# Autodesk Inventor assembly: Piston Feed Platform assy
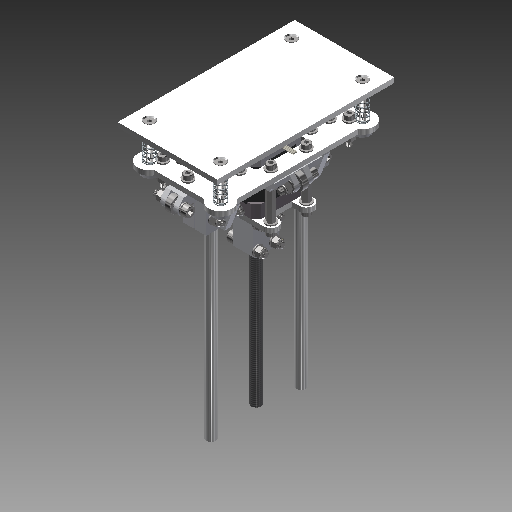
[picture p0: Inventor's stored thumbnail of the model, 512x512]
Saved by Autodesk Inventor 2018 (Build 220112000, 112)
## iProperties
Created: 2017-09-29
Part Number: Piston Feed Platform assy
Document SubType Name: Assembly
Designer: Gabriel Smolnycki
Author: Gabriel Smolnycki
## Documents named in this file (15)
- E:\planb\mechanics\Subassemblies\Piston Feed Platform assy.iam
- E:\planb\mechanics\Piston\Piston Feed Frame.ipt
- E:\planb\mechanics\Subassemblies\Piston Guide assy.iam
- E:\planb\mechanics\Hardware\M4x20 SS SHCS.ipt
- E:\planb\mechanics\Hardware\M4 SS Washer.ipt
- E:\planb\mechanics\Hardware\M4 SS Locknut.ipt
- E:\planb\mechanics\Subassemblies\Piston Wall Guide Wide assy.iam
- E:\planb\mechanics\Subassemblies\Piston Wall Guide Small assy.iam
- E:\planb\mechanics\Piston\Piston Nut Trap.ipt
- E:\planb\mechanics\Piston\Piston Feed Surface.ipt
- E:\planb\mechanics\Hardware\0.375x1.000 Steel Spring (9657K306).ipt
- E:\planb\mechanics\Hardware\M4x40 SS FHSS.ipt
- E:\planb\mechanics\Subassemblies\Piston Motor Holder assy.iam
- E:\planb\mechanics\Hardware\M4x25 SS Standoff FF (94868A045).ipt
- E:\planb\mechanics\Hardware\M4x12 SS SHCS.ipt
## Components (109 placed, 14 different names)
1. Piston Feed Frame:1 — Insert:1, Insert:2, Insert:3, Insert:4, Insert:5, Insert:6, Insert:7, Insert:8, Insert:9, Insert:10, Insert:11, Insert:12, Insert:37, Insert:38, Insert:39, Insert:40, Flush:1, Mate:1, Tangent:1, Mate:4, Flush:2, Tangent:2, Insert:53, Mate:7, Insert:54, Mate:8, Insert:56, Insert:60, Insert:63, Insert:64, Insert:65, Insert:78, Insert:79, Insert:80, Insert:81, Insert:82, Insert:83, Insert:84, Insert:85, Insert:86, Mate:29, Insert:87, Insert:88
2. Piston Guide assy:1 [sub-assembly] — Insert:3, Insert:4, Insert:15, Insert:16, Insert:19, Insert:20
3. Piston Guide assy:2 [sub-assembly] — Insert:1, Insert:2, Insert:13, Insert:14, Insert:17, Insert:18
4. M4x20 SS SHCS:1 — Insert:36
5. M4x20 SS SHCS:2 — Insert:35
6. M4x20 SS SHCS:3 — Insert:32
7. M4x20 SS SHCS:4 — Insert:31
8. M4x20 SS SHCS:5 — Insert:34
9. M4x20 SS SHCS:6 — Insert:33
10. M4x20 SS SHCS:7 — Insert:30
11. M4x20 SS SHCS:8 — Insert:29
12. M4 SS Washer:1 — Insert:18, Insert:24
13. M4 SS Washer:2 — Insert:15, Insert:26
14. M4 SS Washer:3 — Insert:9, Insert:33
15. M4 SS Washer:4 — Insert:7, Insert:35
16. M4 SS Washer:5 — Insert:8, Insert:36
17. M4 SS Washer:6 — Insert:11, Insert:31
18. M4 SS Washer:7 — Insert:16, Insert:25
19. M4 SS Washer:8 — Insert:19, Insert:28
20. M4 SS Washer:9 — Insert:20, Insert:27
21. M4 SS Washer:10 — Insert:17, Insert:22
22. M4 SS Washer:11 — Insert:12, Insert:32
23. M4 SS Washer:12 — Insert:6, Insert:30
24. M4 SS Washer:13 — Insert:10, Insert:34
25. M4 SS Washer:14 — Insert:13, Insert:23
26. M4 SS Washer:15 — Insert:14, Insert:21
27. M4 SS Washer:16 — Insert:5, Insert:29
28. M4 SS Locknut:1 — Insert:21
29. M4 SS Locknut:2 — Insert:22
30. M4 SS Locknut:3 — Insert:24
31. M4 SS Locknut:4 — Insert:23
32. M4 SS Locknut:5 — Insert:28
33. M4 SS Locknut:6 — Insert:27
34. M4 SS Locknut:7 — Insert:26
35. M4 SS Locknut:8 — Insert:25
36. Piston Wall Guide Wide assy:1 [sub-assembly] — Mate:4, Flush:2, Tangent:2, Mate:5, Mate:6
37. Piston Wall Guide Wide assy:2 [sub-assembly] — Flush:1, Mate:1, Tangent:1, Mate:2, Mate:3
38. M4 SS Washer:17 — Mate:5, Insert:92
39. M4 SS Washer:18 — Mate:6, Insert:91
40. M4 SS Washer:19 — Insert:40
41. M4 SS Washer:20 — Insert:39
42. M4 SS Washer:21 — Mate:2, Insert:89
43. M4 SS Washer:22 — Mate:3, Insert:90
44. M4 SS Washer:23 — Insert:38
45. M4 SS Washer:24 — Insert:37
46. M4x20 SS SHCS:9
47. M4x20 SS SHCS:10
48. M4x20 SS SHCS:11
49. M4x20 SS SHCS:12
50. Piston Wall Guide Small assy:1 [sub-assembly] — Insert:54, Mate:8, Insert:55
51. Piston Wall Guide Small assy:2 [sub-assembly] — Insert:53, Mate:7, Insert:59
52. M4 SS Washer:25 — Insert:60, Insert:61
53. M4 SS Washer:26 — Insert:59, Insert:62
54. M4 SS Washer:27 — Insert:56, Insert:57
55. M4 SS Washer:28 — Insert:55, Insert:58
56. M4 SS Locknut:13 — Insert:62
57. M4 SS Locknut:14 — Insert:58
58. M4x20 SS SHCS:13 — Insert:57
59. M4x20 SS SHCS:14 — Insert:61
60. Piston Nut Trap:1 — Mate:9, Flush:3, Mate:10, Insert:63, Insert:66
61. M4 SS Locknut:15 — Insert:67
62. M4 SS Locknut:16 — Mate:9, Flush:3, Mate:10, Insert:64
63. M4 SS Washer:29 — Insert:66, Insert:67
64. M4 SS Washer:30 — Insert:65, Insert:68
65. M4x20 SS SHCS:15 — Insert:68
66. Piston Nut Trap:2 — Insert:80
67. M4 SS Locknut:17
68. M4 SS Locknut:18 — Insert:79
69. M4 SS Washer:31
70. M4 SS Washer:32 — Insert:78
71. M4x20 SS SHCS:16
72. Piston Nut Trap:3 — Insert:82
73. M4 SS Locknut:19
74. M4 SS Locknut:20 — Insert:83
75. M4 SS Washer:33
76. M4 SS Washer:34 — Insert:81
77. M4x20 SS SHCS:17
78. Piston Nut Trap:4 — Insert:85
79. M4 SS Locknut:21
80. M4 SS Locknut:22 — Insert:86
81. M4 SS Washer:35
82. M4 SS Washer:36 — Insert:84
83. M4x20 SS SHCS:18
84. Piston Feed Surface:1 — Mate:17, Mate:18, Mate:19, Mate:20, Mate:21, Mate:22, Mate:23, Mate:24
85. 0.375x1.000 Steel Spring (9657K306):1 — Mate:24, Mate:25
86. 0.375x1.000 Steel Spring (9657K306):2 — Mate:23, Mate:26, Mate:29
87. 0.375x1.000 Steel Spring (9657K306):3 — Mate:22, Mate:27
88. 0.375x1.000 Steel Spring (9657K306):4 — Mate:21, Mate:28
89. M4x40 SS FHSS:1 — Mate:20, Mate:25
90. M4x40 SS FHSS:2 — Mate:19, Mate:26, Insert:88
91. M4x40 SS FHSS:3 — Mate:18, Mate:27, Insert:87
92. M4x40 SS FHSS:4 — Mate:17, Mate:28
93. Piston Motor Holder assy:1 [sub-assembly] — Insert:93, Insert:94, Insert:95, Insert:96, Insert:97, Insert:98, Insert:99, Insert:100
94. M4x25 SS Standoff FF (94868A045):1 — Insert:89, Insert:105
95. M4x25 SS Standoff FF (94868A045):2 — Insert:90
96. M4x25 SS Standoff FF (94868A045):3 — Insert:91, Insert:106
97. M4x25 SS Standoff FF (94868A045):4 — Insert:92
98. M4 SS Washer:37 — Insert:99, Insert:106
99. M4 SS Washer:38 — Insert:97
100. M4 SS Washer:39 — Insert:95, Insert:102
101. M4 SS Washer:40 — Insert:93, Insert:104
102. M4 SS Washer:41 — Insert:100, Insert:105
103. M4 SS Washer:42 — Insert:98
104. M4 SS Washer:43 — Insert:96, Insert:101
105. M4 SS Washer:44 — Insert:94, Insert:103
106. M4x12 SS SHCS:1 — Insert:104
107. M4x12 SS SHCS:2 — Insert:103
108. M4x12 SS SHCS:3 — Insert:102
109. M4x12 SS SHCS:4 — Insert:101
## Relationships (139: Insert 102, Mate 29, Flush 6, Tangent 2)
- Insert:1: Piston Feed Frame:1 ↔ Piston Guide assy:2
- Insert:2: Piston Feed Frame:1 ↔ Piston Guide assy:2
- Insert:3: Piston Feed Frame:1 ↔ Piston Guide assy:1
- Insert:4: Piston Feed Frame:1 ↔ Piston Guide assy:1
- Insert:5: Piston Feed Frame:1 ↔ M4 SS Washer:16
- Insert:6: Piston Feed Frame:1 ↔ M4 SS Washer:12
- Insert:7: Piston Feed Frame:1 ↔ M4 SS Washer:4
- Insert:8: Piston Feed Frame:1 ↔ M4 SS Washer:5
- Insert:9: Piston Feed Frame:1 ↔ M4 SS Washer:3
- Insert:10: Piston Feed Frame:1 ↔ M4 SS Washer:13
- Insert:11: Piston Feed Frame:1 ↔ M4 SS Washer:6
- Insert:12: Piston Feed Frame:1 ↔ M4 SS Washer:11
- Insert:13: Piston Guide assy:2 ↔ M4 SS Washer:14
- Insert:14: Piston Guide assy:2 ↔ M4 SS Washer:15
- Insert:15: Piston Guide assy:1 ↔ M4 SS Washer:2
- Insert:16: Piston Guide assy:1 ↔ M4 SS Washer:7
- Insert:17: Piston Guide assy:2 ↔ M4 SS Washer:10
- Insert:18: Piston Guide assy:2 ↔ M4 SS Washer:1
- Insert:19: Piston Guide assy:1 ↔ M4 SS Washer:8
- Insert:20: Piston Guide assy:1 ↔ M4 SS Washer:9
- Insert:21: M4 SS Washer:15 ↔ M4 SS Locknut:1
- Insert:22: M4 SS Washer:10 ↔ M4 SS Locknut:2
- Insert:23: M4 SS Washer:14 ↔ M4 SS Locknut:4
- Insert:24: M4 SS Washer:1 ↔ M4 SS Locknut:3
- Insert:25: M4 SS Washer:7 ↔ M4 SS Locknut:8
- Insert:26: M4 SS Washer:2 ↔ M4 SS Locknut:7
- Insert:27: M4 SS Washer:9 ↔ M4 SS Locknut:6
- Insert:28: M4 SS Washer:8 ↔ M4 SS Locknut:5
- Insert:29: M4x20 SS SHCS:8 ↔ M4 SS Washer:16
- Insert:30: M4x20 SS SHCS:7 ↔ M4 SS Washer:12
- Insert:31: M4x20 SS SHCS:4 ↔ M4 SS Washer:6
- Insert:32: M4x20 SS SHCS:3 ↔ M4 SS Washer:11
- Insert:33: M4x20 SS SHCS:6 ↔ M4 SS Washer:3
- Insert:34: M4x20 SS SHCS:5 ↔ M4 SS Washer:13
- Insert:35: M4x20 SS SHCS:2 ↔ M4 SS Washer:4
- Insert:36: M4x20 SS SHCS:1 ↔ M4 SS Washer:5
- Insert:37: Piston Feed Frame:1 ↔ M4 SS Washer:24
- Insert:38: Piston Feed Frame:1 ↔ M4 SS Washer:23
- Insert:39: Piston Feed Frame:1 ↔ M4 SS Washer:20
- Insert:40: Piston Feed Frame:1 ↔ M4 SS Washer:19
- Flush:1 (0.825 mm): Piston Feed Frame:1 ↔ Piston Wall Guide Wide assy:2
- Mate:1: Piston Feed Frame:1 ↔ Piston Wall Guide Wide assy:2
- Tangent:1: Piston Feed Frame:1 ↔ Piston Wall Guide Wide assy:2
- [Insert]: M4 SS Washer:24 ↔ M4x20 SS SHCS:9
- [Insert]: M4 SS Washer:23 ↔ M4x20 SS SHCS:10
- Mate:2: Piston Wall Guide Wide assy:2 ↔ M4 SS Washer:21
- [Insert]: M4 SS Washer:21 ↔ M4x20 SS SHCS:9
- Mate:3: Piston Wall Guide Wide assy:2 ↔ M4 SS Washer:22
- [Insert]: M4 SS Washer:22 ↔ M4x20 SS SHCS:10
- Mate:4: Piston Feed Frame:1 ↔ Piston Wall Guide Wide assy:1
- Flush:2 (0.825 mm): Piston Feed Frame:1 ↔ Piston Wall Guide Wide assy:1
- Tangent:2: Piston Feed Frame:1 ↔ Piston Wall Guide Wide assy:1
- [Insert]: M4 SS Washer:20 ↔ M4x20 SS SHCS:11
- [Insert]: M4 SS Washer:19 ↔ M4x20 SS SHCS:12
- Mate:5: Piston Wall Guide Wide assy:1 ↔ M4 SS Washer:17
- Mate:6: Piston Wall Guide Wide assy:1 ↔ M4 SS Washer:18
- [Insert]: M4 SS Washer:17 ↔ M4x20 SS SHCS:11
- [Insert]: M4 SS Washer:18 ↔ M4x20 SS SHCS:12
- Insert:53: Piston Feed Frame:1 ↔ Piston Wall Guide Small assy:2
- Mate:7: Piston Feed Frame:1 ↔ Piston Wall Guide Small assy:2
- Insert:54: Piston Feed Frame:1 ↔ Piston Wall Guide Small assy:1
- Mate:8: Piston Feed Frame:1 ↔ Piston Wall Guide Small assy:1
- Insert:55: Piston Wall Guide Small assy:1 ↔ M4 SS Washer:28
- Insert:56: Piston Feed Frame:1 ↔ M4 SS Washer:27
- Insert:57: M4 SS Washer:27 ↔ M4x20 SS SHCS:13
- Insert:58: M4 SS Washer:28 ↔ M4 SS Locknut:14
- Insert:59: Piston Wall Guide Small assy:2 ↔ M4 SS Washer:26
- Insert:60: Piston Feed Frame:1 ↔ M4 SS Washer:25
- Insert:61: M4 SS Washer:25 ↔ M4x20 SS SHCS:14
- Insert:62: M4 SS Washer:26 ↔ M4 SS Locknut:13
- Mate:9: Piston Nut Trap:1 ↔ M4 SS Locknut:16
- Flush:3: Piston Nut Trap:1 ↔ M4 SS Locknut:16
- Mate:10: Piston Nut Trap:1 ↔ M4 SS Locknut:16
- Insert:63: Piston Feed Frame:1 ↔ Piston Nut Trap:1
- Insert:64: Piston Feed Frame:1 ↔ M4 SS Locknut:16
- Insert:65: Piston Feed Frame:1 ↔ M4 SS Washer:30
- Insert:66: Piston Nut Trap:1 ↔ M4 SS Washer:29
- Insert:67: M4 SS Locknut:15 ↔ M4 SS Washer:29
- Insert:68: M4 SS Washer:30 ↔ M4x20 SS SHCS:15
- [Mate]: Piston Nut Trap:2 ↔ M4 SS Locknut:18
- [Flush]: Piston Nut Trap:2 ↔ M4 SS Locknut:18
- [Mate]: Piston Nut Trap:2 ↔ M4 SS Locknut:18
- [Insert]: Piston Nut Trap:2 ↔ M4 SS Washer:31
- [Insert]: M4 SS Locknut:17 ↔ M4 SS Washer:31
- [Insert]: M4 SS Washer:32 ↔ M4x20 SS SHCS:16
- [Mate]: Piston Nut Trap:3 ↔ M4 SS Locknut:20
- [Flush]: Piston Nut Trap:3 ↔ M4 SS Locknut:20
- [Mate]: Piston Nut Trap:3 ↔ M4 SS Locknut:20
- [Insert]: Piston Nut Trap:3 ↔ M4 SS Washer:33
- [Insert]: M4 SS Locknut:19 ↔ M4 SS Washer:33
- [Insert]: M4 SS Washer:34 ↔ M4x20 SS SHCS:17
- [Mate]: Piston Nut Trap:4 ↔ M4 SS Locknut:22
- [Flush]: Piston Nut Trap:4 ↔ M4 SS Locknut:22
- [Mate]: Piston Nut Trap:4 ↔ M4 SS Locknut:22
- [Insert]: Piston Nut Trap:4 ↔ M4 SS Washer:35
- [Insert]: M4 SS Locknut:21 ↔ M4 SS Washer:35
- [Insert]: M4 SS Washer:36 ↔ M4x20 SS SHCS:18
- Insert:78: Piston Feed Frame:1 ↔ M4 SS Washer:32
- Insert:79: Piston Feed Frame:1 ↔ M4 SS Locknut:18
- Insert:80: Piston Feed Frame:1 ↔ Piston Nut Trap:2
- Insert:81: Piston Feed Frame:1 ↔ M4 SS Washer:34
- Insert:82: Piston Feed Frame:1 ↔ Piston Nut Trap:3
- Insert:83: Piston Feed Frame:1 ↔ M4 SS Locknut:20
- Insert:84: Piston Feed Frame:1 ↔ M4 SS Washer:36
- Insert:85: Piston Feed Frame:1 ↔ Piston Nut Trap:4
- Insert:86: Piston Feed Frame:1 ↔ M4 SS Locknut:22
- Mate:17: Piston Feed Surface:1 ↔ M4x40 SS FHSS:4
- Mate:18: Piston Feed Surface:1 ↔ M4x40 SS FHSS:3
- Mate:19: Piston Feed Surface:1 ↔ M4x40 SS FHSS:2
- Mate:20: Piston Feed Surface:1 ↔ M4x40 SS FHSS:1
- Mate:21: Piston Feed Surface:1 ↔ 0.375x1.000 Steel Spring (9657K306):4
- Mate:22: Piston Feed Surface:1 ↔ 0.375x1.000 Steel Spring (9657K306):3
- Mate:23: Piston Feed Surface:1 ↔ 0.375x1.000 Steel Spring (9657K306):2
- Mate:24: Piston Feed Surface:1 ↔ 0.375x1.000 Steel Spring (9657K306):1
- Mate:25: 0.375x1.000 Steel Spring (9657K306):1 ↔ M4x40 SS FHSS:1
- Mate:26: 0.375x1.000 Steel Spring (9657K306):2 ↔ M4x40 SS FHSS:2
- Mate:27: 0.375x1.000 Steel Spring (9657K306):3 ↔ M4x40 SS FHSS:3
- Mate:28: 0.375x1.000 Steel Spring (9657K306):4 ↔ M4x40 SS FHSS:4
- Mate:29: Piston Feed Frame:1 ↔ 0.375x1.000 Steel Spring (9657K306):2
- Insert:87: Piston Feed Frame:1 ↔ M4x40 SS FHSS:3
- Insert:88: Piston Feed Frame:1 ↔ M4x40 SS FHSS:2
- Insert:89: M4 SS Washer:21 ↔ M4x25 SS Standoff FF (94868A045):1
- Insert:90: M4 SS Washer:22 ↔ M4x25 SS Standoff FF (94868A045):2
- Insert:91: M4 SS Washer:18 ↔ M4x25 SS Standoff FF (94868A045):3
- Insert:92: M4 SS Washer:17 ↔ M4x25 SS Standoff FF (94868A045):4
- Insert:93: Piston Motor Holder assy:1 ↔ M4 SS Washer:40
- Insert:94: Piston Motor Holder assy:1 ↔ M4 SS Washer:44
- Insert:95: Piston Motor Holder assy:1 ↔ M4 SS Washer:39
- Insert:96: Piston Motor Holder assy:1 ↔ M4 SS Washer:43
- Insert:97: Piston Motor Holder assy:1 ↔ M4 SS Washer:38
- Insert:98: Piston Motor Holder assy:1 ↔ M4 SS Washer:42
- Insert:99: Piston Motor Holder assy:1 ↔ M4 SS Washer:37
- Insert:100: Piston Motor Holder assy:1 ↔ M4 SS Washer:41
- Insert:101: M4 SS Washer:43 ↔ M4x12 SS SHCS:4
- Insert:102: M4 SS Washer:39 ↔ M4x12 SS SHCS:3
- Insert:103: M4 SS Washer:44 ↔ M4x12 SS SHCS:2
- Insert:104: M4 SS Washer:40 ↔ M4x12 SS SHCS:1
- Insert:105: M4x25 SS Standoff FF (94868A045):1 ↔ M4 SS Washer:41
- Insert:106: M4x25 SS Standoff FF (94868A045):3 ↔ M4 SS Washer:37
## Named parameters: d137_d134 = 0 mm, d138_d135 = 0 mm, d139_d136 = 0 mm, d140_d128 = 0 mm, d141_d129 = 0 mm, d142_d130 = 0 mm, d143_d134 = 0 mm, d144_d135 = 0 mm, d145_d136 = 0 mm, d146_d128 = 0 mm, d147_d129 = 0 mm, d148_d130 = 0 mm, d149_d134 = 0 mm, d150_d135 = 0 mm, d151_d136 = 0 mm, d152_d128 = 0 mm, d153_d129 = 0 mm, d154_d130 = 0 mm
